# Autodesk Inventor assembly: Exstra håndtag
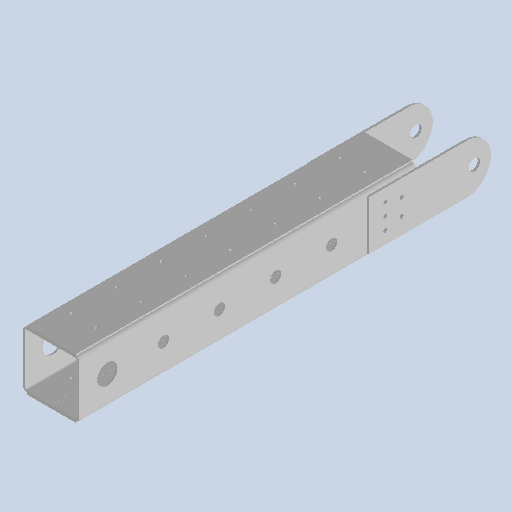
[picture p0: Inventor's stored thumbnail of the model, 512x512]
Saved by Autodesk Inventor 2022 (Build 260153000, 153)
## iProperties
Created: 2022-04-12
Part Number: Exstra håndtag
Document SubType Name: Weldment
Designer: Patrick
Weld Material: Welded Aluminum-6061
Author: Patrick
## Documents named in this file (4)
- C:\Users\patri\OneDrive - Syddansk Universitet\2. Semester Master\Mekaniske Elementer\Mini Project\2020-10-23\Workspaces\Workspace\Extra_Beam\Exstra håndtag.iam
- C:\Users\patri\OneDrive - Syddansk Universitet\2. Semester Master\Mekaniske Elementer\Mini Project\2020-10-23\Workspaces\Workspace\Extra_Beam\Extra led trækhåndtag.ipt
- C:\Users\patri\OneDrive - Syddansk Universitet\2. Semester Master\Mekaniske Elementer\Mini Project\2020-10-23\Workspaces\Workspace\Extra_Beam\Beslag ekstra håndtag.ipt
- C:\Users\patri\OneDrive - Syddansk Universitet\2. Semester Master\Mekaniske Elementer\Mini Project\2020-10-23\Workspaces\Workspace\Extra_Beam\Samle_plade.ipt
## Components (6 placed, 3 different names)
1. Extra led trækhåndtag:1 — Rigid:4, Rigid:5, Mate:4
2. Extra led trækhåndtag:2 — Rigid:4, Rigid:6, Mate:1, Mate:2, Flush:1, Mate:3, Flush:2
3. Beslag ekstra håndtag:1 — Rigid:5
4. Beslag ekstra håndtag:2 — Rigid:6
5. Samle_plade:1 — Mate:1, Mate:2, Flush:1
6. Samle_plade:2 — Mate:3, Flush:2, Mate:4
## Relationships (9: Mate 4, WeldJoint 3, Flush 2)
- Rigid:4 [WeldJoint]: Extra led trækhåndtag:1 ↔ Extra led trækhåndtag:2
- Rigid:5 [WeldJoint]: Extra led trækhåndtag:1 ↔ Beslag ekstra håndtag:1
- Rigid:6 [WeldJoint]: Extra led trækhåndtag:2 ↔ Beslag ekstra håndtag:2
- Mate:1: Extra led trækhåndtag:2 ↔ Samle_plade:1
- Mate:2: Extra led trækhåndtag:2 ↔ Samle_plade:1
- Flush:1: Extra led trækhåndtag:2 ↔ Samle_plade:1
- Mate:3: Extra led trækhåndtag:2 ↔ Samle_plade:2
- Flush:2: Extra led trækhåndtag:2 ↔ Samle_plade:2
- Mate:4: Extra led trækhåndtag:1 ↔ Samle_plade:2
